# Autodesk Inventor assembly: AX12
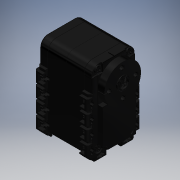
[picture p0: Inventor's stored thumbnail of the model, 180x180]
Saved by Autodesk Inventor 2017 (Build 210142000, 142)
## iProperties
Created: 2010-02-01
Part Number: AX12
Document SubType Name: Assembly
Designer: Andrew
Translation Standard: STEP AP203
File Name: AX12_Fixed.STEP
Preprocessor: SolidWorks 2010
Postprocessor: Build: 254, Release: 2008 - Date: Fri 03/23/2007
Sent Units: MILLIMETERS
Uncertainty: 1e-05
Author: Andrew
## Documents named in this file (4)
- C:\Users\franc\Desktop\EsialRobotik\Mecanique\composants\AX12\AX12.iam
- C:\Users\franc\Desktop\EsialRobotik\Mecanique\composants\AX12\ax12_wheel.ipt
- C:\Users\franc\Desktop\EsialRobotik\Mecanique\composants\AX12\ax12_box.ipt
- C:\Users\franc\Desktop\EsialRobotik\Mecanique\composants\AX12\ax12_cog.ipt
## Components (3 placed, 3 different names)
1. ax12_wheel:1 — Insert:1
2. ax12_box:1 — Insert:1
3. ax12_cog:1
## Relationships (1: Insert 1)
- Insert:1: ax12_wheel:1 ↔ ax12_box:1
